# Autodesk Inventor assembly: 4138T531_Gas Spring (1)
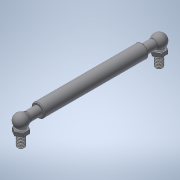
[picture p0: Inventor's stored thumbnail of the model, 180x180]
Saved by Autodesk Inventor 2020 (Build 240168000, 168)
## iProperties
Created: 2022-01-30
Part Number: 4138T531_Gas Spring (1)
Document SubType Name: Assembly
Designer: mavericks
Author: mavericks
## Documents named in this file (6)
- T:\EIT\2022 Rapid React\COMMON PARTS\MCMASTER\Gas spring\4138T531_Gas Spring (1).iam
- T:\EIT\2022 Rapid React\COMMON PARTS\MCMASTER\Gas spring\Solid1_1.ipt
- T:\EIT\2022 Rapid React\COMMON PARTS\MCMASTER\Gas spring\Solid2_1.ipt
- T:\EIT\2022 Rapid React\COMMON PARTS\MCMASTER\Gas spring\Solid3_1.ipt
- T:\EIT\2022 Rapid React\COMMON PARTS\MCMASTER\Gas spring\Solid4_1.ipt
- T:\EIT\2022 Rapid React\COMMON PARTS\MCMASTER\Gas spring\Solid7_1.ipt
## Components (5 placed, 5 different names)
1. Solid1_1:1
2. Solid2_1:1 — Angle:1, Mate:3
3. Solid3_1:1 — Mate:1, Mate:2, Tangent:1
4. Solid4_1:1 — Mate:1
5. Solid7_1:1 — Mate:2, Tangent:1, Angle:1, Mate:3
## Relationships (5: Mate 3, Tangent 1, Angle 1)
- Mate:1: Solid3_1:1 ↔ Solid4_1:1
- Mate:2: Solid3_1:1 ↔ Solid7_1:1
- Tangent:1: Solid3_1:1 ↔ Solid7_1:1
- Angle:1 (180 deg): Solid2_1:1 ↔ Solid7_1:1
- Mate:3: Solid2_1:1 ↔ Solid7_1:1
